# Autodesk Inventor assembly: canon_reservoir
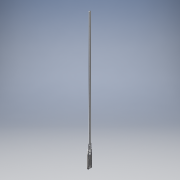
[picture p0: Inventor's stored thumbnail of the model, 180x180]
Saved by Autodesk Inventor 2019 (Build 230136000, 136)
## iProperties
Created: 2019-03-25
Part Number: canon_reservoir
Material: Générique
Document SubType Name: Assembly
Designer: theor
Mass: 702.15 g
Surface Area: 1447.39 cm^2
Volume: 182.547 cm^3
Density: 3.8464 g/cm^3
Author: theor
## Documents named in this file (7)
- C:\dev\projects\ace\ace-git\ACE-FP 12 Prot 2\canon_reservoir.iam
- C:\dev\projects\ace\ace-git\ACE-FP 12 Prot 2\tube_reservoir.ipt
- C:\dev\projects\ace\ace-git\ACE-FP 12 Prot 2\reservoir_jointure.ipt
- C:\dev\projects\ace\ace-git\ACE-FP 12 Prot 2\support_douille.ipt
- C:\dev\projects\ace\ace-git\ACE-FP 12 Prot 2\tube_canon.ipt
- C:\dev\projects\ace\ace-git\ACE-FP 12 Prot 2\blocage_recule_support_douille.ipt
- C:\dev\projects\ace\ace-git\ACE-FP 12 Prot 2\piston_reservoir.ipt
## Components (6 placed, 6 different names)
1. tube_reservoir:1 — Placage:1, Placage:2, Placage:7
2. reservoir_jointure:1 — Placage:1, Placage:2, Placage:3
3. support_douille:1 — Placage:3, Placage:4, Placage:5
4. tube_canon:1 — Placage:4, Placage:5, Placage:6
5. blocage_recule_support_douille:1 — Placage:6
6. piston_reservoir:1 — Placage:7
## Relationships (7: Mate 7)
- Placage:1 [Mate]: tube_reservoir:1 ↔ reservoir_jointure:1
- Placage:2 [Mate]: tube_reservoir:1 ↔ reservoir_jointure:1
- Placage:3 [Mate]: reservoir_jointure:1 ↔ support_douille:1
- Placage:4 [Mate]: support_douille:1 ↔ tube_canon:1
- Placage:5 [Mate]: support_douille:1 ↔ tube_canon:1
- Placage:6 [Mate]: tube_canon:1 ↔ blocage_recule_support_douille:1
- Placage:7 [Mate]: tube_reservoir:1 ↔ piston_reservoir:1
